# Autodesk Inventor assembly: RobotMK2
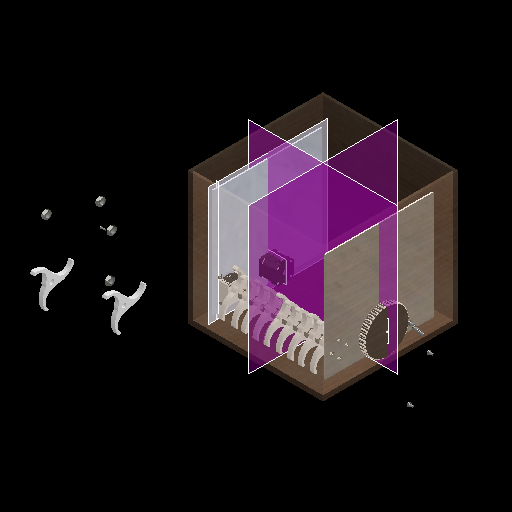
[picture p0: Inventor's stored thumbnail of the model, 512x512]
Saved by Autodesk Inventor 2025 (Build 290162000, 162)
## iProperties
Created: 2025-01-19
Part Number: RobotMK2
Document SubType Name: Assembly
Designer: Trevor
Author: Trevor
## Documents named in this file (17)
- C:\Users\Trevor\Documents\GitHub\USA-Robotic-Club-2024\assests\RobotMK2.iam
- C:\Users\Trevor\Documents\GitHub\USA-Robotic-Club-2024\assests\RightALPanel.ipt
- C:\Users\Trevor\Documents\GitHub\USA-Robotic-Club-2024\assests\LeftALPanel.ipt
- C:\Users\Trevor\Documents\GitHub\USA-Robotic-Club-2024\assests\RobotWheelMK1.ipt
- C:\Users\Trevor\Documents\GitHub\USA-Robotic-Club-2024\assests\Robot Box.ipt
- C:\Users\Trevor\Documents\GitHub\USA-Robotic-Club-2024\assests\17hm08-1204s-nema17-pancake-21mm-1.snapshot.2\17HM08-1204S Nema17 Pancake 21mm\17HM08-1204S Nema17 Pancake 21mm.ipt
- C:\Users\Trevor\Documents\GitHub\USA-Robotic-Club-2024\assests\stepperonline-nema-17-1.snapshot.1\Stepper Motor\Stepper Motor.ipt
- C:\Users\Trevor\Documents\GitHub\USA-Robotic-Club-2024\assests\RodMK3.ipt
- C:\Users\Trevor\Documents\GitHub\USA-Robotic-Club-2024\assests\Combine mk5.ipt
- C:\Users\Trevor\Documents\GitHub\USA-Robotic-Club-2024\assests\bearing-10mm-2.snapshot.2\PMG(Si)\PMG(Si).ipt
- C:\Users\Trevor\Documents\Inventor\Content Center Files\R2025\en-US\DIN 934\DIN 934 - M10 x 1.ipt
- C:\Users\Trevor\Documents\GitHub\USA-Robotic-Club-2024\assests\PanpackeMotorMountMK2.ipt
- C:\Users\Trevor\Documents\GitHub\USA-Robotic-Club-2024\assests\BearingMountMK2.ipt
- C:\Users\Trevor\Documents\Inventor\Content Center Files\R2025\en-US\ANSI B18.3.4M(1)\ANSI B18.3.4M - M5 x 0.8 x 8(2).ipt
- C:\Users\Trevor\Documents\Inventor\Content Center Files\R2025\en-US\DIN 934\DIN 934 - M5 x 0.8.ipt
- C:\Users\Trevor\Documents\Inventor\Content Center Files\R2025\en-US\ANSI B18.3.4M(1)\ANSI B18.3.4M - M3 x 0.5 x 10(2).ipt
- C:\Users\Trevor\Documents\Inventor\Content Center Files\R2025\en-US\ANSI B18.3.4M(1)\ANSI B18.3.4M - M5 x 0.8 x 10(2).ipt
## Components (76 placed, 16 different names)
1. Robot Box:1 — Mate:1, Mate:2, Mate:3, Mate:4, Mate:5, Mate:6, Mate:7, Flush:3, Flush:4, Mate:12
2. RobotWheelMK1:1 — Mate:2, Mate:3, Mate:4, Flush:1, Mate:8
3. RobotWheelMK1:2 — Mate:5, Mate:6, Mate:7, Mate:10
4. RightALPanel:1 — Flush:5, Mate:9, Mate:21, Flush:11, Mate:74, Mate:76, Mate:77, Mate:79, Mate:81, Mate:82, Mate:83, Mate:88, Mate:91, Mate:92, Mate:93, Mate:94, Mate:95, Mate:96, Mate:97
5. LeftAlPanel:1 — Flush:6, Mate:11, Mate:17, Flush:7, Flush:10, Mate:98, Mate:99, Mate:100, Mate:101, Mate:102, Mate:103, Mate:104, Mate:105, Mate:106, Mate:107, Mate:108, Mate:116, Mate:117, Mate:118, Mate:122, Mate:124
6. Stepper Motor:1 — Mate:8, Mate:9, Mate:13, Mate:90
7. Stepper Motor:2 — Mate:10, Mate:11, Mate:12, Mate:13
8. RodMK3:1 — Mate:18, Mate:19, Mate:20, Mate:22, Mate:24, Mate:26, Mate:28, Mate:29, Mate:30, Mate:31, Mate:33, Mate:34, Mate:38, Mate:39, Mate:43, Mate:44, Mate:48, Mate:50, Mate:52, Mate:54, Mate:55, Mate:58, Mate:60, Mate:61, Mate:64, Mate:66, Mate:67, Mate:70, Mate:72
9. 17HM08-1204S Nema17 Pancake 21mm:1 — Mate:17, Mate:18, Mate:19, Flush:8, Mate:23, Flush:9
10. PMG(Si):1 — Mate:20, Mate:21
11. Combine mk5:1 — Mate:22, Mate:23, Mate:25
12. DIN 934 - replaced by DIN EN 24032/28673/28674 M10 x 1:1 — Mate:24, Mate:25, Mate:27
13. DIN 934 - replaced by DIN EN 24032/28673/28674 M10 x 1:2 — Mate:26, Mate:27, Mate:32
14. DIN 934 - replaced by DIN EN 24032/28673/28674 M10 x 1:4 — Mate:48, Mate:49, Mate:51
15. DIN 934 - replaced by DIN EN 24032/28673/28674 M10 x 1:3 — Mate:33, Mate:35, Mate:36
16. DIN 934 - replaced by DIN EN 24032/28673/28674 M10 x 1:5 — Mate:34, Mate:36, Mate:37
17. DIN 934 - replaced by DIN EN 24032/28673/28674 M10 x 1:6 — Mate:38, Mate:40, Mate:41
18. DIN 934 - replaced by DIN EN 24032/28673/28674 M10 x 1:7 — Mate:50, Mate:51, Mate:53
19. DIN 934 - replaced by DIN EN 24032/28673/28674 M10 x 1:8 — Mate:44, Mate:46, Mate:47
20. DIN 934 - replaced by DIN EN 24032/28673/28674 M10 x 1:9 — Mate:43, Mate:45, Mate:46
21. DIN 934 - replaced by DIN EN 24032/28673/28674 M10 x 1:10 — Mate:39, Mate:41, Mate:42
22. DIN 934 - replaced by DIN EN 24032/28673/28674 M10 x 1:11 — Mate:60, Mate:62, Mate:63
23. DIN 934 - replaced by DIN EN 24032/28673/28674 M10 x 1:12 — Mate:66, Mate:68, Mate:69
24. Combine mk5:2 — Mate:28, Mate:32, Mate:35
25. Combine mk5:3 — Mate:29, Mate:37, Mate:40
26. Combine mk5:4 — Mate:30, Mate:42, Mate:45
27. Combine mk5:5 — Mate:31, Mate:47, Mate:49
28. Combine mk5:6
29. Combine mk5:7 — Mate:70, Mate:71, Mate:73
30. Combine mk5:8 — Mate:58, Mate:59, Mate:62
31. Combine mk5:9 — Mate:64, Mate:65, Mate:68
32. Combine mk5:10
33. Combine mk5:11 — Mate:52, Mate:53, Mate:56
34. DIN 934 - replaced by DIN EN 24032/28673/28674 M10 x 1:13 — Mate:61, Mate:63, Mate:65
35. DIN 934 - replaced by DIN EN 24032/28673/28674 M10 x 1:14 — Mate:67, Mate:69, Mate:71
36. DIN 934 - replaced by DIN EN 24032/28673/28674 M10 x 1:15
37. DIN 934 - replaced by DIN EN 24032/28673/28674 M10 x 1:16
38. DIN 934 - replaced by DIN EN 24032/28673/28674 M10 x 1:17 — Mate:54, Mate:56, Mate:57
39. DIN 934 - replaced by DIN EN 24032/28673/28674 M10 x 1:18 — Mate:55, Mate:57, Mate:59
40. DIN 934 - replaced by DIN EN 24032/28673/28674 M10 x 1:19 — Mate:72, Mate:73
41. DIN 934 - replaced by DIN EN 24032/28673/28674 M10 x 1:20
42. DIN 934 - replaced by DIN EN 24032/28673/28674 M10 x 1:21
43. PanpackeMotorMountMK2:1 — Flush:9, Flush:10, Mate:109, Mate:110, Mate:111, Mate:112, Mate:113, Mate:114, Mate:115
44. BearingMountMK2:1 — Flush:11, Mate:75, Mate:78, Mate:80, Mate:126
45. Broached Hexagon Socket Button Head Cap Screw - Metric M5 x 0.8 x 10:8 — Mate:74, Mate:75, Mate:84
46. Broached Hexagon Socket Button Head Cap Screw - Metric M5 x 0.8 x 10:9 — Mate:76, Mate:85, Mate:126
47. Broached Hexagon Socket Button Head Cap Screw - Metric M5 x 0.8 x 8:3
48. Broached Hexagon Socket Button Head Cap Screw - Metric M5 x 0.8 x 10:1 — Mate:106, Mate:115, Mate:125
49. Broached Hexagon Socket Button Head Cap Screw - Metric M5 x 0.8 x 10:7 — Mate:77, Mate:78, Mate:89
50. Broached Hexagon Socket Button Head Cap Screw - Metric M5 x 0.8 x 8:6
51. Broached Hexagon Socket Button Head Cap Screw - Metric M5 x 0.8 x 8:7
52. Broached Hexagon Socket Button Head Cap Screw - Metric M5 x 0.8 x 10:6 — Mate:79, Mate:80, Mate:87
53. Broached Hexagon Socket Button Head Cap Screw - Metric M5 x 0.8 x 8:9
54. Broached Hexagon Socket Button Head Cap Screw - Metric M5 x 0.8 x 8:10
55. DIN 934 - replaced by DIN EN 24032/28673/28674 M5:1 — Mate:82, Mate:85
56. DIN 934 - replaced by DIN EN 24032/28673/28674 M5:2 — Mate:81, Mate:84
57. DIN 934 - replaced by DIN EN 24032/28673/28674 M5:4 — Mate:83, Mate:87
58. DIN 934 - replaced by DIN EN 24032/28673/28674 M5:5 — Mate:88, Mate:89
59. Broached Hexagon Socket Button Head Cap Screw - Metric M3 x 0.5 x 10:1 — Mate:94, Mate:96
60. Broached Hexagon Socket Button Head Cap Screw - Metric M3 x 0.5 x 10:2 — Mate:93, Mate:95
61. Broached Hexagon Socket Button Head Cap Screw - Metric M3 x 0.5 x 10:3
62. Broached Hexagon Socket Button Head Cap Screw - Metric M3 x 0.5 x 10:4 — Mate:92, Mate:97
63. Broached Hexagon Socket Button Head Cap Screw - Metric M3 x 0.5 x 10:5 — Mate:90, Mate:91
64. Broached Hexagon Socket Button Head Cap Screw - Metric M3 x 0.5 x 10:7 — Mate:98, Mate:102
65. Broached Hexagon Socket Button Head Cap Screw - Metric M3 x 0.5 x 10:8 — Mate:99, Mate:104
66. Broached Hexagon Socket Button Head Cap Screw - Metric M3 x 0.5 x 10:9 — Mate:100, Mate:105
67. Broached Hexagon Socket Button Head Cap Screw - Metric M3 x 0.5 x 10:10 — Mate:101, Mate:103
68. Broached Hexagon Socket Button Head Cap Screw - Metric M5 x 0.8 x 10:2 — Mate:107, Mate:114, Mate:121
69. Broached Hexagon Socket Button Head Cap Screw - Metric M5 x 0.8 x 10:3 — Mate:108, Mate:113, Mate:123
70. Broached Hexagon Socket Button Head Cap Screw - Metric M5 x 0.8 x 10:4 — Mate:109, Mate:112, Mate:119
71. Broached Hexagon Socket Button Head Cap Screw - Metric M5 x 0.8 x 10:5 — Mate:110, Mate:111, Mate:120
72. DIN 934 - replaced by DIN EN 24032/28673/28674 M5:6 — Mate:118, Mate:121
73. DIN 934 - replaced by DIN EN 24032/28673/28674 M5:7 — Mate:117, Mate:119
74. DIN 934 - replaced by DIN EN 24032/28673/28674 M5:8 — Mate:122, Mate:123
75. DIN 934 - replaced by DIN EN 24032/28673/28674 M5:10 — Mate:116, Mate:120
76. DIN 934 - replaced by DIN EN 24032/28673/28674 M5:11 — Mate:124, Mate:125
## Relationships (132: Mate 122, Flush 10)
- Mate:1: Robot Box:1
- Mate:2: Robot Box:1 ↔ RobotWheelMK1:1
- Mate:3 (2 mm): Robot Box:1 ↔ RobotWheelMK1:1
- Mate:4: Robot Box:1 ↔ RobotWheelMK1:1
- Mate:5: Robot Box:1 ↔ RobotWheelMK1:2
- Mate:6 (2 mm): Robot Box:1 ↔ RobotWheelMK1:2
- Mate:7: Robot Box:1 ↔ RobotWheelMK1:2
- Flush:1 (2 mm): RobotWheelMK1:1
- Flush:3 (20 mm): Robot Box:1
- Flush:4 (20 mm): Robot Box:1
- Flush:5: RightALPanel:1
- Flush:6: LeftAlPanel:1
- Mate:8: RobotWheelMK1:1 ↔ Stepper Motor:1
- Mate:9: RightALPanel:1 ↔ Stepper Motor:1
- Mate:10: RobotWheelMK1:2 ↔ Stepper Motor:2
- Mate:11: LeftAlPanel:1 ↔ Stepper Motor:2
- Mate:12: Robot Box:1 ↔ Stepper Motor:2
- Mate:13: Stepper Motor:1 ↔ Stepper Motor:2
- Mate:17: LeftAlPanel:1 ↔ 17HM08-1204S Nema17 Pancake 21mm:1
- Mate:18: RodMK3:1 ↔ 17HM08-1204S Nema17 Pancake 21mm:1
- Mate:19: RodMK3:1 ↔ 17HM08-1204S Nema17 Pancake 21mm:1
- Flush:7 (-10 mm): LeftAlPanel:1
- Flush:8: 17HM08-1204S Nema17 Pancake 21mm:1
- Mate:20: RodMK3:1 ↔ PMG(Si):1
- Mate:21: RightALPanel:1 ↔ PMG(Si):1
- Mate:22: RodMK3:1 ↔ Combine mk5:1
- Mate:23: 17HM08-1204S Nema17 Pancake 21mm:1 ↔ Combine mk5:1
- Mate:24: RodMK3:1 ↔ DIN 934 - replaced by DIN EN 24032/28673/28674 M10 x 1:1
- Mate:25: Combine mk5:1 ↔ DIN 934 - replaced by DIN EN 24032/28673/28674 M10 x 1:1
- Mate:26: RodMK3:1 ↔ DIN 934 - replaced by DIN EN 24032/28673/28674 M10 x 1:2
- Mate:27: DIN 934 - replaced by DIN EN 24032/28673/28674 M10 x 1:1 ↔ DIN 934 - replaced by DIN EN 24032/28673/28674 M10 x 1:2
- Mate:28: RodMK3:1 ↔ Combine mk5:2
- Mate:29: RodMK3:1 ↔ Combine mk5:3
- Mate:30: RodMK3:1 ↔ Combine mk5:4
- Mate:31: RodMK3:1 ↔ Combine mk5:5
- Mate:32: DIN 934 - replaced by DIN EN 24032/28673/28674 M10 x 1:2 ↔ Combine mk5:2
- Mate:33: RodMK3:1 ↔ DIN 934 - replaced by DIN EN 24032/28673/28674 M10 x 1:3
- Mate:34: RodMK3:1 ↔ DIN 934 - replaced by DIN EN 24032/28673/28674 M10 x 1:5
- Mate:35: DIN 934 - replaced by DIN EN 24032/28673/28674 M10 x 1:3 ↔ Combine mk5:2
- Mate:36: DIN 934 - replaced by DIN EN 24032/28673/28674 M10 x 1:3 ↔ DIN 934 - replaced by DIN EN 24032/28673/28674 M10 x 1:5
- Mate:37: DIN 934 - replaced by DIN EN 24032/28673/28674 M10 x 1:5 ↔ Combine mk5:3
- Mate:38: RodMK3:1 ↔ DIN 934 - replaced by DIN EN 24032/28673/28674 M10 x 1:6
- Mate:39: RodMK3:1 ↔ DIN 934 - replaced by DIN EN 24032/28673/28674 M10 x 1:10
- Mate:40: DIN 934 - replaced by DIN EN 24032/28673/28674 M10 x 1:6 ↔ Combine mk5:3
- Mate:41: DIN 934 - replaced by DIN EN 24032/28673/28674 M10 x 1:6 ↔ DIN 934 - replaced by DIN EN 24032/28673/28674 M10 x 1:10
- Mate:42: DIN 934 - replaced by DIN EN 24032/28673/28674 M10 x 1:10 ↔ Combine mk5:4
- Mate:43: RodMK3:1 ↔ DIN 934 - replaced by DIN EN 24032/28673/28674 M10 x 1:9
- Mate:44: RodMK3:1 ↔ DIN 934 - replaced by DIN EN 24032/28673/28674 M10 x 1:8
- Mate:45: DIN 934 - replaced by DIN EN 24032/28673/28674 M10 x 1:9 ↔ Combine mk5:4
- Mate:46: DIN 934 - replaced by DIN EN 24032/28673/28674 M10 x 1:8 ↔ DIN 934 - replaced by DIN EN 24032/28673/28674 M10 x 1:9
- Mate:47: DIN 934 - replaced by DIN EN 24032/28673/28674 M10 x 1:8 ↔ Combine mk5:5
- Mate:48: RodMK3:1 ↔ DIN 934 - replaced by DIN EN 24032/28673/28674 M10 x 1:4
- Mate:49: DIN 934 - replaced by DIN EN 24032/28673/28674 M10 x 1:4 ↔ Combine mk5:5
- Mate:50: RodMK3:1 ↔ DIN 934 - replaced by DIN EN 24032/28673/28674 M10 x 1:7
- Mate:51: DIN 934 - replaced by DIN EN 24032/28673/28674 M10 x 1:4 ↔ DIN 934 - replaced by DIN EN 24032/28673/28674 M10 x 1:7
- Mate:52: RodMK3:1 ↔ Combine mk5:11
- Mate:53: DIN 934 - replaced by DIN EN 24032/28673/28674 M10 x 1:7 ↔ Combine mk5:11
- Mate:54: RodMK3:1 ↔ DIN 934 - replaced by DIN EN 24032/28673/28674 M10 x 1:17
- Mate:55: RodMK3:1 ↔ DIN 934 - replaced by DIN EN 24032/28673/28674 M10 x 1:18
- Mate:56: Combine mk5:11 ↔ DIN 934 - replaced by DIN EN 24032/28673/28674 M10 x 1:17
- Mate:57: DIN 934 - replaced by DIN EN 24032/28673/28674 M10 x 1:17 ↔ DIN 934 - replaced by DIN EN 24032/28673/28674 M10 x 1:18
- Mate:58: RodMK3:1 ↔ Combine mk5:8
- Mate:59: Combine mk5:8 ↔ DIN 934 - replaced by DIN EN 24032/28673/28674 M10 x 1:18
- Mate:60: RodMK3:1 ↔ DIN 934 - replaced by DIN EN 24032/28673/28674 M10 x 1:11
- Mate:61: RodMK3:1 ↔ DIN 934 - replaced by DIN EN 24032/28673/28674 M10 x 1:13
- Mate:62: DIN 934 - replaced by DIN EN 24032/28673/28674 M10 x 1:11 ↔ Combine mk5:8
- Mate:63: DIN 934 - replaced by DIN EN 24032/28673/28674 M10 x 1:11 ↔ DIN 934 - replaced by DIN EN 24032/28673/28674 M10 x 1:13
- Mate:64: RodMK3:1 ↔ Combine mk5:9
- Mate:65: Combine mk5:9 ↔ DIN 934 - replaced by DIN EN 24032/28673/28674 M10 x 1:13
- Mate:66: RodMK3:1 ↔ DIN 934 - replaced by DIN EN 24032/28673/28674 M10 x 1:12
- Mate:67: RodMK3:1 ↔ DIN 934 - replaced by DIN EN 24032/28673/28674 M10 x 1:14
- Mate:68: DIN 934 - replaced by DIN EN 24032/28673/28674 M10 x 1:12 ↔ Combine mk5:9
- Mate:69: DIN 934 - replaced by DIN EN 24032/28673/28674 M10 x 1:12 ↔ DIN 934 - replaced by DIN EN 24032/28673/28674 M10 x 1:14
- Mate:70: RodMK3:1 ↔ Combine mk5:7
- Mate:71: Combine mk5:7 ↔ DIN 934 - replaced by DIN EN 24032/28673/28674 M10 x 1:14
- Mate:72: RodMK3:1 ↔ DIN 934 - replaced by DIN EN 24032/28673/28674 M10 x 1:19
- Mate:73: Combine mk5:7 ↔ DIN 934 - replaced by DIN EN 24032/28673/28674 M10 x 1:19
- Flush:9: 17HM08-1204S Nema17 Pancake 21mm:1 ↔ PanpackeMotorMountMK2:1
- Flush:10: LeftAlPanel:1 ↔ PanpackeMotorMountMK2:1
- Flush:11: RightALPanel:1 ↔ BearingMountMK2:1
- Mate:74: RightALPanel:1 ↔ Broached Hexagon Socket Button Head Cap Screw - Metric M5 x 0.8 x 10:8
- Mate:75: BearingMountMK2:1 ↔ Broached Hexagon Socket Button Head Cap Screw - Metric M5 x 0.8 x 10:8
- Mate:76: RightALPanel:1 ↔ Broached Hexagon Socket Button Head Cap Screw - Metric M5 x 0.8 x 10:9
- Mate:77: RightALPanel:1 ↔ Broached Hexagon Socket Button Head Cap Screw - Metric M5 x 0.8 x 10:7
- Mate:78: BearingMountMK2:1 ↔ Broached Hexagon Socket Button Head Cap Screw - Metric M5 x 0.8 x 10:7
- Mate:79: RightALPanel:1 ↔ Broached Hexagon Socket Button Head Cap Screw - Metric M5 x 0.8 x 10:6
- Mate:80: BearingMountMK2:1 ↔ Broached Hexagon Socket Button Head Cap Screw - Metric M5 x 0.8 x 10:6
- Mate:81: RightALPanel:1 ↔ DIN 934 - replaced by DIN EN 24032/28673/28674 M5:2
- Mate:82: RightALPanel:1 ↔ DIN 934 - replaced by DIN EN 24032/28673/28674 M5:1
- Mate:83: RightALPanel:1 ↔ DIN 934 - replaced by DIN EN 24032/28673/28674 M5:4
- Mate:84: Broached Hexagon Socket Button Head Cap Screw - Metric M5 x 0.8 x 10:8 ↔ DIN 934 - replaced by DIN EN 24032/28673/28674 M5:2
- Mate:85: Broached Hexagon Socket Button Head Cap Screw - Metric M5 x 0.8 x 10:9 ↔ DIN 934 - replaced by DIN EN 24032/28673/28674 M5:1
- Mate:87: Broached Hexagon Socket Button Head Cap Screw - Metric M5 x 0.8 x 10:6 ↔ DIN 934 - replaced by DIN EN 24032/28673/28674 M5:4
- Mate:88: RightALPanel:1 ↔ DIN 934 - replaced by DIN EN 24032/28673/28674 M5:5
- Mate:89: Broached Hexagon Socket Button Head Cap Screw - Metric M5 x 0.8 x 10:7 ↔ DIN 934 - replaced by DIN EN 24032/28673/28674 M5:5
- Mate:90: Stepper Motor:1 ↔ Broached Hexagon Socket Button Head Cap Screw - Metric M3 x 0.5 x 10:5
- Mate:91: RightALPanel:1 ↔ Broached Hexagon Socket Button Head Cap Screw - Metric M3 x 0.5 x 10:5
- Mate:92: RightALPanel:1 ↔ Broached Hexagon Socket Button Head Cap Screw - Metric M3 x 0.5 x 10:4
- Mate:93: RightALPanel:1 ↔ Broached Hexagon Socket Button Head Cap Screw - Metric M3 x 0.5 x 10:2
- Mate:94: RightALPanel:1 ↔ Broached Hexagon Socket Button Head Cap Screw - Metric M3 x 0.5 x 10:1
- Mate:95: RightALPanel:1 ↔ Broached Hexagon Socket Button Head Cap Screw - Metric M3 x 0.5 x 10:2
- Mate:96: RightALPanel:1 ↔ Broached Hexagon Socket Button Head Cap Screw - Metric M3 x 0.5 x 10:1
- Mate:97: RightALPanel:1 ↔ Broached Hexagon Socket Button Head Cap Screw - Metric M3 x 0.5 x 10:4
- Mate:98: LeftAlPanel:1 ↔ Broached Hexagon Socket Button Head Cap Screw - Metric M3 x 0.5 x 10:7
- Mate:99: LeftAlPanel:1 ↔ Broached Hexagon Socket Button Head Cap Screw - Metric M3 x 0.5 x 10:8
- Mate:100: LeftAlPanel:1 ↔ Broached Hexagon Socket Button Head Cap Screw - Metric M3 x 0.5 x 10:9
- Mate:101: LeftAlPanel:1 ↔ Broached Hexagon Socket Button Head Cap Screw - Metric M3 x 0.5 x 10:10
- Mate:102: LeftAlPanel:1 ↔ Broached Hexagon Socket Button Head Cap Screw - Metric M3 x 0.5 x 10:7
- Mate:103: LeftAlPanel:1 ↔ Broached Hexagon Socket Button Head Cap Screw - Metric M3 x 0.5 x 10:10
- Mate:104: LeftAlPanel:1 ↔ Broached Hexagon Socket Button Head Cap Screw - Metric M3 x 0.5 x 10:8
- Mate:105: LeftAlPanel:1 ↔ Broached Hexagon Socket Button Head Cap Screw - Metric M3 x 0.5 x 10:9
- Mate:106: LeftAlPanel:1 ↔ Broached Hexagon Socket Button Head Cap Screw - Metric M5 x 0.8 x 10:1
- Mate:107: LeftAlPanel:1 ↔ Broached Hexagon Socket Button Head Cap Screw - Metric M5 x 0.8 x 10:2
- Mate:108: LeftAlPanel:1 ↔ Broached Hexagon Socket Button Head Cap Screw - Metric M5 x 0.8 x 10:3
- Mate:109: PanpackeMotorMountMK2:1 ↔ Broached Hexagon Socket Button Head Cap Screw - Metric M5 x 0.8 x 10:4
- Mate:110: PanpackeMotorMountMK2:1 ↔ Broached Hexagon Socket Button Head Cap Screw - Metric M5 x 0.8 x 10:5
- Mate:111: PanpackeMotorMountMK2:1 ↔ Broached Hexagon Socket Button Head Cap Screw - Metric M5 x 0.8 x 10:5
- Mate:112: PanpackeMotorMountMK2:1 ↔ Broached Hexagon Socket Button Head Cap Screw - Metric M5 x 0.8 x 10:4
- Mate:113: PanpackeMotorMountMK2:1 ↔ Broached Hexagon Socket Button Head Cap Screw - Metric M5 x 0.8 x 10:3
- Mate:114: PanpackeMotorMountMK2:1 ↔ Broached Hexagon Socket Button Head Cap Screw - Metric M5 x 0.8 x 10:2
- Mate:115: PanpackeMotorMountMK2:1 ↔ Broached Hexagon Socket Button Head Cap Screw - Metric M5 x 0.8 x 10:1
- Mate:116: LeftAlPanel:1 ↔ DIN 934 - replaced by DIN EN 24032/28673/28674 M5:10
- Mate:117: LeftAlPanel:1 ↔ DIN 934 - replaced by DIN EN 24032/28673/28674 M5:7
- Mate:118: LeftAlPanel:1 ↔ DIN 934 - replaced by DIN EN 24032/28673/28674 M5:6
- Mate:119: Broached Hexagon Socket Button Head Cap Screw - Metric M5 x 0.8 x 10:4 ↔ DIN 934 - replaced by DIN EN 24032/28673/28674 M5:7
- Mate:120: Broached Hexagon Socket Button Head Cap Screw - Metric M5 x 0.8 x 10:5 ↔ DIN 934 - replaced by DIN EN 24032/28673/28674 M5:10
- Mate:121: Broached Hexagon Socket Button Head Cap Screw - Metric M5 x 0.8 x 10:2 ↔ DIN 934 - replaced by DIN EN 24032/28673/28674 M5:6
- Mate:122: LeftAlPanel:1 ↔ DIN 934 - replaced by DIN EN 24032/28673/28674 M5:8
- Mate:123: Broached Hexagon Socket Button Head Cap Screw - Metric M5 x 0.8 x 10:3 ↔ DIN 934 - replaced by DIN EN 24032/28673/28674 M5:8
- Mate:124: LeftAlPanel:1 ↔ DIN 934 - replaced by DIN EN 24032/28673/28674 M5:11
- Mate:125: Broached Hexagon Socket Button Head Cap Screw - Metric M5 x 0.8 x 10:1 ↔ DIN 934 - replaced by DIN EN 24032/28673/28674 M5:11
- Mate:126: BearingMountMK2:1 ↔ Broached Hexagon Socket Button Head Cap Screw - Metric M5 x 0.8 x 10:9
